# Autodesk Inventor assembly: 2021-01-001_o
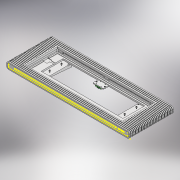
[picture p0: Inventor's stored thumbnail of the model, 180x180]
Saved by Autodesk Inventor 2020.2 (Build 242310000, 310)
## iProperties
Created: 2021-04-25
Part Number: 2021-01-001_o
Document SubType Name: Assembly
Designer: carso
Author: carso
## Documents named in this file (75)
- P:\Carson Wright Design Projects\KB__kbd-2600\KBD2600 MANUFACTURING ASSETS\CAD FILES\IPT\2021-01-001_o.iam
- P:\Carson Wright Design Projects\KB__kbd-2600\FINAL\2021-01-002.ipt
- P:\Carson Wright Design Projects\KB__kbd-2600\FINAL\2021-01-006.ipt
- P:\Carson Wright Design Projects\KB__kbd-2600\FINAL\2021-01-011.ipt
- P:\Carson Wright Design Projects\KB__kbd-2600\FINAL\2021-01-013_pp.ipt
- P:\Carson Wright Design Projects\KB__kbd-2600\FINAL\2021-01-017_pp.ipt
- P:\Carson Wright Design Projects\KB__kbd-2600\FINAL\2021-01-015_pp.ipt
- P:\Carson Wright Design Projects\KB__kbd-2600\FINAL\2021-01-003.ipt
- P:\Carson Wright Design Projects\KB__kbd-2600\FINAL\2021-01-021_pp.ipt
- P:\Carson Wright Design Projects\KB__kbd-2600\FINAL\2021-01-019_pp.ipt
- P:\Carson Wright Design Projects\KB__kbd-2600\FINAL\2021-01-018_pp.ipt
- P:\Carson Wright Design Projects\KB__kbd-2600\FINAL\2021-01-016.ipt
- P:\Carson Wright Design Projects\KB__kbd-2600\FINAL\2021-01-022.iam
- P:\Carson Wright Design Projects\KB__kbd-2600\FINAL\2021-01-020_pp.ipt
- P:\Carson Wright Design Projects\KB__kbd-2600\FINAL\2021-01-007.ipt
- P:\Carson Wright Design Projects\KB__kbd-2600\FINAL\2021-01-008.ipt
- P:\Assets\Keycaps\CherryMX-master\CherryMX-master-updated\CherryMX-master\r1 legended\STP\Esc.ipt
- P:\Assets\Keycaps\CherryMX-master\CherryMX-master-updated\CherryMX-master\r1 legended\STP\1_NEW.ipt
- P:\Assets\Keycaps\CherryMX-master\CherryMX-master-updated\CherryMX-master\r1 legended\STP\2.ipt
- P:\Assets\Keycaps\CherryMX-master\CherryMX-master-updated\CherryMX-master\r1 legended\STP\4.ipt
- P:\Assets\Keycaps\CherryMX-master\CherryMX-master-updated\CherryMX-master\r1 legended\STP\5_NEW.ipt
- P:\Assets\Keycaps\CherryMX-master\CherryMX-master-updated\CherryMX-master\r1 legended\STP\3 ansi.ipt
- P:\Assets\Keycaps\CherryMX-master\CherryMX-master-updated\CherryMX-master\r1 legended\STP\6.ipt
- P:\Assets\Keycaps\CherryMX-master\CherryMX-master-updated\CherryMX-master\r1 legended\STP\7.ipt
- P:\Assets\Keycaps\CherryMX-master\CherryMX-master-updated\CherryMX-master\r1 legended\STP\8.ipt
- P:\Assets\Keycaps\CherryMX-master\CherryMX-master-updated\CherryMX-master\r1 legended\STP\9.ipt
- P:\Assets\Keycaps\CherryMX-master\CherryMX-master-updated\CherryMX-master\r1 legended\STP\-.ipt
- P:\Assets\Keycaps\CherryMX-master\CherryMX-master-updated\CherryMX-master\r1 legended\STP\0.ipt
- P:\Assets\Keycaps\CherryMX-master\CherryMX-master-updated\CherryMX-master\r1 legended\STP\=.ipt
- P:\Assets\Keycaps\CherryMX-master\CherryMX-master-updated\CherryMX-master\r1 legended\STP\TILDE.ipt
- P:\Assets\Keycaps\CherryMX-master\CherryMX-master-updated\CherryMX-master\r1 legended\STP\pipe.ipt
- P:\Assets\Keycaps\CherryMX-master\CherryMX-master-updated\CherryMX-master\r2 legended\STP\Q.ipt
- P:\Assets\Keycaps\CherryMX-master\CherryMX-master-updated\CherryMX-master\r2 legended\STP\W.ipt
- P:\Assets\Keycaps\CherryMX-master\CherryMX-master-updated\CherryMX-master\r2 legended\STP\E.ipt
- P:\Assets\Keycaps\CherryMX-master\CherryMX-master-updated\CherryMX-master\r2 legended\STP\R.ipt
- P:\Assets\Keycaps\CherryMX-master\CherryMX-master-updated\CherryMX-master\r2 legended\STP\T.ipt
- P:\Assets\Keycaps\CherryMX-master\CherryMX-master-updated\CherryMX-master\r2 legended\STP\Y.ipt
- P:\Assets\Keycaps\CherryMX-master\CherryMX-master-updated\CherryMX-master\r2 legended\STP\U.ipt
- P:\Assets\Keycaps\CherryMX-master\CherryMX-master-updated\CherryMX-master\r2 legended\STP\I.ipt
- P:\Assets\Keycaps\CherryMX-master\CherryMX-master-updated\CherryMX-master\r2 legended\STP\O.ipt
- P:\Assets\Keycaps\CherryMX-master\CherryMX-master-updated\CherryMX-master\r2 legended\STP\P.ipt
- P:\Assets\Keycaps\CherryMX-master\CherryMX-master-updated\CherryMX-master\r2 legended\STP\OPEN BRACKETS.ipt
- P:\Assets\Keycaps\CherryMX-master\CherryMX-master-updated\CherryMX-master\r2 legended\STP\CLOSE BRACKETS.ipt
- P:\Assets\Keycaps\CherryMX-master\CherryMX-master-updated\CherryMX-master\r2 legended\STP\15\Backspace text.ipt
- P:\Assets\Keycaps\CherryMX-master\CherryMX-master-updated\CherryMX-master\r2 legended\STP\15\Tab text.ipt
- P:\Assets\Keycaps\CherryMX-master\CherryMX-master-updated\CherryMX-master\r3 legended\STP\175\Control.ipt
- P:\Assets\Keycaps\CherryMX-master\CherryMX-master-updated\CherryMX-master\r3 legended\STP\A.ipt
- P:\Assets\Keycaps\CherryMX-master\CherryMX-master-updated\CherryMX-master\r3 legended\STP\S.ipt
- P:\Assets\Keycaps\CherryMX-master\CherryMX-master-updated\CherryMX-master\r3 legended\STP\D.ipt
- P:\Assets\Keycaps\CherryMX-master\CherryMX-master-updated\CherryMX-master\r3 legended\STP\F_homing_bar.ipt
- P:\Assets\Keycaps\CherryMX-master\CherryMX-master-updated\CherryMX-master\r3 legended\STP\G.ipt
- P:\Assets\Keycaps\CherryMX-master\CherryMX-master-updated\CherryMX-master\r3 legended\STP\H.ipt
- P:\Assets\Keycaps\CherryMX-master\CherryMX-master-updated\CherryMX-master\r3 legended\STP\J_homing_bar.ipt
- P:\Assets\Keycaps\CherryMX-master\CherryMX-master-updated\CherryMX-master\r3 legended\STP\K.ipt
- P:\Assets\Keycaps\CherryMX-master\CherryMX-master-updated\CherryMX-master\r3 legended\STP\L.ipt
- P:\Assets\Keycaps\CherryMX-master\CherryMX-master-updated\CherryMX-master\r3 legended\STP\COLONS.ipt
- P:\Assets\Keycaps\CherryMX-master\CherryMX-master-updated\CherryMX-master\r3 legended\STP\quotes.ipt
- P:\Assets\Keycaps\CherryMX-master\CherryMX-master\r3 legended\STP\225\Enter Text 225 Fixed.ipt
- P:\Assets\Keycaps\CherryMX-master\CherryMX-master\r4 legended\STP\225\Shift text.ipt
- P:\Assets\Keycaps\CherryMX-master\CherryMX-master\r4 legended\STP\Z.ipt
- P:\Assets\Keycaps\CherryMX-master\CherryMX-master\r4 legended\STP\X.ipt
- P:\Assets\Keycaps\CherryMX-master\CherryMX-master\r4 legended\STP\C.ipt
- P:\Assets\Keycaps\CherryMX-master\CherryMX-master\r4 legended\STP\V.ipt
- P:\Assets\Keycaps\CherryMX-master\CherryMX-master\r4 legended\STP\B.ipt
- P:\Assets\Keycaps\CherryMX-master\CherryMX-master\r4 legended\STP\N.ipt
- P:\Assets\Keycaps\CherryMX-master\CherryMX-master\r4 legended\STP\M.ipt
- P:\Assets\Keycaps\CherryMX-master\CherryMX-master\r4 legended\STP\COMMA.ipt
- P:\Assets\Keycaps\CherryMX-master\CherryMX-master\r4 legended\STP\FULL STOP.ipt
- P:\Assets\Keycaps\CherryMX-master\CherryMX-master\r4 legended\STP\Fn.ipt
- P:\Assets\Keycaps\CherryMX-master\CherryMX-master\r4 legended\STP\FORWARD SLASH.ipt
- P:\Assets\Keycaps\CherryMX-master\CherryMX-master\r4 legended\STP\175\Shift short text.ipt
- P:\Assets\Keycaps\CherryMX-master\CherryMX-master\STEP\r4\r4_150.ipt
- P:\Assets\Keycaps\CherryMX-master\CherryMX-master-updated\CherryMX-master\r4 legended\STP\CODE.ipt
- P:\Assets\Keycaps\CherryMX-master\CherryMX-master-updated\CherryMX-master\r4 legended\STP\15\Alt.ipt
- P:\Assets\Keycaps\CherryMX-master\CherryMX-master-updated\CherryMX-master\STEP\r4\r4_700.ipt
## Components (102 placed, 74 different names)
1. 2021-01-002:1 — Mate:34, Mate:35, Mate:36, Mate:37, Mate:38, Mate:39, Mate:40, Mate:41, Mate:42, Mate:43, Mate:44, Mate:45, Mate:53, Mate:54, Mate:55, Mate:57, Mate:59, Mate:61, Mate:63, Mate:65, Mate:67, Mate:68, Mate:69, Mate:70, Mate:71, Mate:73, Mate:75, Mate:77, Mate:79, Mate:80, Mate:81, Mate:82, Mate:83, Mate:84, Mate:85, Mate:86, Mate:87, Mate:88, Mate:89, Mate:90
2. 2021-01-006:1 — Mate:46, Mate:47, Mate:48, Mate:49, Mate:51, Mate:68, Mate:69, Mate:70, Mate:116, Mate:117, Mate:118, Mate:119
3. 2021-01-011:1 — Mate:4, Mate:5, Mate:6, Mate:46, Mate:47, Mate:48, Mate:50, Mate:52
4. 2021-01-013_pp:1 — Mate:4, Mate:5, Mate:6, Mate:7, Mate:8, Mate:9, Mate:10, Mate:11, Mate:12, Mate:13, Mate:14
5. 2021-01-017_pp:1 — Mate:7, Mate:8
6. 2021-01-017_pp:2 — Mate:9, Mate:10
7. 2021-01-017_pp:3 — Mate:13, Mate:14
8. 2021-01-017_pp:4 — Mate:11, Mate:12
9. 2021-01-015_pp:1 — Mate:34, Mate:35, Mate:36
10. 2021-01-015_pp:2 — Mate:37, Mate:38, Mate:39
11. 2021-01-015_pp:3 — Mate:43, Mate:44, Mate:45
12. 2021-01-015_pp:4 — Mate:40, Mate:41, Mate:42
13. 2021-01-003:1 — Mate:53, Mate:54, Mate:55, Mate:56, Mate:58, Mate:60, Mate:62, Mate:64, Mate:66, Mate:92, Mate:93, Mate:94, Mate:95, Mate:96, Mate:97, Mate:98, Mate:99, Mate:100, Mate:101, Mate:110, Mate:111, Mate:112, Mate:113, Mate:114, Mate:115
14. 2021-01-021_pp:1 — Mate:51, Mate:52
15. 2021-01-021_pp:2 — Mate:49, Mate:50
16. 2021-01-019_pp:1 — Mate:58, Mate:59
17. 2021-01-019_pp:2 — Mate:56, Mate:57
18. 2021-01-019_pp:3 — Mate:66, Mate:67
19. 2021-01-019_pp:4 — Mate:64, Mate:65
20. 2021-01-019_pp:5 — Mate:60, Mate:61
21. 2021-01-019_pp:6 — Mate:62, Mate:63
22. 2021-01-018_pp:1 — Mate:71, Mate:116
23. 2021-01-018_pp:2 — Mate:73, Mate:117
24. 2021-01-018_pp:3 — Mate:75, Mate:118
25. 2021-01-018_pp:4 — Mate:77, Mate:119
26. 2021-01-016:1 — Mate:88, Mate:89, Mate:90
27. 2021-01-016:2 — Mate:82, Mate:83, Mate:84
28. 2021-01-016:3 — Mate:79, Mate:80, Mate:81
29. 2021-01-016:4 — Mate:85, Mate:86, Mate:87, Mate:91
30. 2021-01-022:1 [sub-assembly] — Mate:91, Mate:92, Mate:93, Mate:120, Mate:121, Mate:122, Mate:123, Mate:124, Mate:125, Mate:128, Mate:129, Mate:130, Mate:131, Mate:132, Mate:133, Mate:134, Mate:135, Mate:136, Mate:137, Mate:138, Mate:139, Mate:140, Mate:141, Mate:142, Mate:143, Mate:144, Mate:145, Mate:146, Mate:147, Mate:148, Mate:149, Mate:150, Mate:151, Mate:154, Mate:155, Mate:156, Mate:157, Mate:158, Mate:159, Mate:160, Mate:161, Mate:162, Mate:163, Mate:164, Mate:165, Mate:166, Mate:167, Mate:168, Mate:169, Mate:170, Mate:171, Mate:172, Mate:173, Mate:174, Mate:175, Mate:176, Mate:177, Mate:178, Mate:179, Mate:180, Mate:181, Mate:182, Mate:183, Mate:184, Mate:185, Mate:186, Mate:187, Mate:188, Mate:189, Mate:190, Mate:191, Mate:192, Mate:193, Mate:194, Mate:195, Mate:196, Mate:197, Mate:198, Mate:199, Mate:200, Mate:201, Mate:202, Mate:203, Mate:204, Mate:205, Mate:206, Mate:207, Mate:208, Mate:209, Mate:210, Mate:211, Mate:212, Mate:213, Mate:214, Mate:215, Mate:216, Mate:217, Mate:218, Mate:219, Mate:220, Mate:221, Mate:222, Mate:223, Mate:224, Mate:225, Mate:226, Mate:227, Mate:228, Mate:229, Mate:230, Mate:231, Mate:232, Mate:233, Mate:234, Mate:235, Mate:236, Mate:237, Mate:238, Mate:239, Mate:240, Mate:241, Mate:242, Mate:243, Mate:244, Mate:245, Mate:246, Mate:247
31. 2021-01-020_pp:1 — Mate:94, Mate:95
32. 2021-01-020_pp:2 — Mate:96, Mate:97
33. 2021-01-020_pp:3 — Mate:100, Mate:101
34. 2021-01-020_pp:4 — Mate:98, Mate:99
35. 2021-01-007:1 — Mate:106, Mate:107, Mate:108, Mate:109, Mate:113, Mate:114, Mate:115
36. 2021-01-008:1 — Mate:102, Mate:103, Mate:104, Mate:105, Mate:110, Mate:111, Mate:112
37. 2021-01-020_pp:5 — Mate:102, Mate:103
38. 2021-01-020_pp:6 — Mate:108, Mate:109
39. 2021-01-020_pp:7 — Mate:106, Mate:107
40. 2021-01-020_pp:8 — Mate:104, Mate:105
41. Esc:1 — Mate:120, Mate:121
42. 1_NEW:1 — Mate:122, Mate:123
43. 2:1 — Mate:124, Mate:125
44. 4:1 — Mate:128, Mate:129
45. 5_NEW:1 — Mate:132, Mate:133
46. 3 ansi:1 — Mate:130, Mate:131
47. 6:1 — Mate:134, Mate:135
48. 7:1 — Mate:136, Mate:137
49. 8:1 — Mate:138, Mate:139
50. 9:1 — Mate:140, Mate:141
51. -:1 — Mate:144, Mate:145
52. 0:1 — Mate:142, Mate:143
53. =:1 — Mate:146, Mate:147
54. TILDE:1 — Mate:150, Mate:151
55. pipe:1 — Mate:148, Mate:149
56. Q:1 — Mate:154, Mate:155
57. W:1 — Mate:156, Mate:157
58. E:1 — Mate:158, Mate:159
59. R:1 — Mate:160, Mate:161
60. T:1 — Mate:162, Mate:163
61. Y:1 — Mate:164, Mate:165
62. U:1 — Mate:166, Mate:167
63. I:1 — Mate:168, Mate:169
64. O:1 — Mate:170, Mate:171
65. P:1 — Mate:172, Mate:173
66. OPEN BRACKETS:1 — Mate:174, Mate:175
67. CLOSE BRACKETS:1 — Mate:176, Mate:177
68. Backspace text:1 — Mate:178, Mate:179
69. Tab text:1 — Mate:180, Mate:181
70. Control:1 — Mate:182, Mate:183
71. A:1 — Mate:184, Mate:185
72. S:1 — Mate:186, Mate:187
73. D:1 — Mate:188, Mate:189
74. F_homing_bar:1 — Mate:190, Mate:191
75. G:1 — Mate:192, Mate:193
76. H:1 — Mate:194, Mate:195
77. J_homing_bar:1 — Mate:196, Mate:197
78. K:1 — Mate:198, Mate:199
79. L:1 — Mate:200, Mate:201
80. COLONS:1 — Mate:202, Mate:203
81. quotes:1 — Mate:204, Mate:205
82. Enter Text 225 Fixed:1 — Mate:206, Mate:207
83. Shift text:1 — Mate:208, Mate:209
84. Z:1 — Mate:210, Mate:211
85. X:1 — Mate:212, Mate:213
86. C:1 — Mate:214, Mate:215
87. V:1 — Mate:216, Mate:217
88. B:1 — Mate:218, Mate:219
89. N:1 — Mate:222, Mate:223
90. M:1 — Mate:220, Mate:221
91. COMMA:1 — Mate:224, Mate:225
92. FULL STOP:1 — Mate:226, Mate:227
93. Fn:1 — Mate:230, Mate:231
94. FORWARD SLASH:1 — Mate:228, Mate:229
95. Shift short text:1 — Mate:232, Mate:233
96. r4_150:1 — Mate:234, Mate:235
97. r4_150:2 — Mate:236, Mate:237
98. CODE:1 — Mate:238, Mate:239
99. CODE:2 — Mate:240, Mate:241
100. Alt:1 — Mate:242, Mate:243
101. Alt:2 — Mate:244, Mate:245
102. r4_700:1 — Mate:246, Mate:247
## Relationships (217: Mate 217)
- Mate:4: 2021-01-011:1 ↔ 2021-01-013_pp:1
- Mate:5: 2021-01-011:1 ↔ 2021-01-013_pp:1
- Mate:6: 2021-01-011:1 ↔ 2021-01-013_pp:1
- Mate:7: 2021-01-013_pp:1 ↔ 2021-01-017_pp:1
- Mate:8: 2021-01-013_pp:1 ↔ 2021-01-017_pp:1
- Mate:9: 2021-01-013_pp:1 ↔ 2021-01-017_pp:2
- Mate:10: 2021-01-013_pp:1 ↔ 2021-01-017_pp:2
- Mate:11: 2021-01-013_pp:1 ↔ 2021-01-017_pp:4
- Mate:12: 2021-01-013_pp:1 ↔ 2021-01-017_pp:4
- Mate:13: 2021-01-013_pp:1 ↔ 2021-01-017_pp:3
- Mate:14: 2021-01-013_pp:1 ↔ 2021-01-017_pp:3
- Mate:34 (0.1 mm): 2021-01-002:1 ↔ 2021-01-015_pp:1
- Mate:35: 2021-01-002:1 ↔ 2021-01-015_pp:1
- Mate:36: 2021-01-002:1 ↔ 2021-01-015_pp:1
- Mate:37 (0.1 mm): 2021-01-002:1 ↔ 2021-01-015_pp:2
- Mate:38: 2021-01-002:1 ↔ 2021-01-015_pp:2
- Mate:39: 2021-01-002:1 ↔ 2021-01-015_pp:2
- Mate:40 (0.1 mm): 2021-01-002:1 ↔ 2021-01-015_pp:4
- Mate:41: 2021-01-002:1 ↔ 2021-01-015_pp:4
- Mate:42: 2021-01-002:1 ↔ 2021-01-015_pp:4
- Mate:43 (0.1 mm): 2021-01-002:1 ↔ 2021-01-015_pp:3
- Mate:44: 2021-01-002:1 ↔ 2021-01-015_pp:3
- Mate:45: 2021-01-002:1 ↔ 2021-01-015_pp:3
- Mate:46: 2021-01-006:1 ↔ 2021-01-011:1
- Mate:47: 2021-01-006:1 ↔ 2021-01-011:1
- Mate:48: 2021-01-006:1 ↔ 2021-01-011:1
- Mate:49: 2021-01-006:1 ↔ 2021-01-021_pp:2
- Mate:50: 2021-01-011:1 ↔ 2021-01-021_pp:2
- Mate:51: 2021-01-006:1 ↔ 2021-01-021_pp:1
- Mate:52: 2021-01-011:1 ↔ 2021-01-021_pp:1
- Mate:53: 2021-01-002:1 ↔ 2021-01-003:1
- Mate:54: 2021-01-002:1 ↔ 2021-01-003:1
- Mate:55: 2021-01-002:1 ↔ 2021-01-003:1
- Mate:56: 2021-01-003:1 ↔ 2021-01-019_pp:2
- Mate:57: 2021-01-002:1 ↔ 2021-01-019_pp:2
- Mate:58: 2021-01-003:1 ↔ 2021-01-019_pp:1
- Mate:59: 2021-01-002:1 ↔ 2021-01-019_pp:1
- Mate:60: 2021-01-003:1 ↔ 2021-01-019_pp:5
- Mate:61: 2021-01-002:1 ↔ 2021-01-019_pp:5
- Mate:62: 2021-01-003:1 ↔ 2021-01-019_pp:6
- Mate:63: 2021-01-002:1 ↔ 2021-01-019_pp:6
- Mate:64: 2021-01-003:1 ↔ 2021-01-019_pp:4
- Mate:65: 2021-01-002:1 ↔ 2021-01-019_pp:4
- Mate:66: 2021-01-003:1 ↔ 2021-01-019_pp:3
- Mate:67: 2021-01-002:1 ↔ 2021-01-019_pp:3
- Mate:68: 2021-01-002:1 ↔ 2021-01-006:1
- Mate:69: 2021-01-002:1 ↔ 2021-01-006:1
- Mate:70: 2021-01-002:1 ↔ 2021-01-006:1
- Mate:71: 2021-01-002:1 ↔ 2021-01-018_pp:1
- Mate:73: 2021-01-002:1 ↔ 2021-01-018_pp:2
- Mate:75: 2021-01-002:1 ↔ 2021-01-018_pp:3
- Mate:77: 2021-01-002:1 ↔ 2021-01-018_pp:4
- Mate:79: 2021-01-002:1 ↔ 2021-01-016:3
- Mate:80: 2021-01-002:1 ↔ 2021-01-016:3
- Mate:81: 2021-01-002:1 ↔ 2021-01-016:3
- Mate:82: 2021-01-002:1 ↔ 2021-01-016:2
- Mate:83: 2021-01-002:1 ↔ 2021-01-016:2
- Mate:84: 2021-01-002:1 ↔ 2021-01-016:2
- Mate:85: 2021-01-002:1 ↔ 2021-01-016:4
- Mate:86: 2021-01-002:1 ↔ 2021-01-016:4
- Mate:87: 2021-01-002:1 ↔ 2021-01-016:4
- Mate:88: 2021-01-002:1 ↔ 2021-01-016:1
- Mate:89: 2021-01-002:1 ↔ 2021-01-016:1
- Mate:90: 2021-01-002:1 ↔ 2021-01-016:1
- Mate:91: 2021-01-016:4 ↔ 2021-01-022:1
- Mate:92 (0.2 mm): 2021-01-003:1 ↔ 2021-01-022:1
- Mate:93 (0.2 mm): 2021-01-003:1 ↔ 2021-01-022:1
- Mate:94: 2021-01-003:1 ↔ 2021-01-020_pp:1
- Mate:95: 2021-01-003:1 ↔ 2021-01-020_pp:1
- Mate:96: 2021-01-003:1 ↔ 2021-01-020_pp:2
- Mate:97: 2021-01-003:1 ↔ 2021-01-020_pp:2
- Mate:98: 2021-01-003:1 ↔ 2021-01-020_pp:4
- Mate:99: 2021-01-003:1 ↔ 2021-01-020_pp:4
- Mate:100: 2021-01-003:1 ↔ 2021-01-020_pp:3
- Mate:101: 2021-01-003:1 ↔ 2021-01-020_pp:3
- Mate:102: 2021-01-008:1 ↔ 2021-01-020_pp:5
- Mate:103: 2021-01-008:1 ↔ 2021-01-020_pp:5
- Mate:104: 2021-01-008:1 ↔ 2021-01-020_pp:8
- Mate:105: 2021-01-008:1 ↔ 2021-01-020_pp:8
- Mate:106: 2021-01-007:1 ↔ 2021-01-020_pp:7
- Mate:107: 2021-01-007:1 ↔ 2021-01-020_pp:7
- Mate:108: 2021-01-007:1 ↔ 2021-01-020_pp:6
- Mate:109: 2021-01-007:1 ↔ 2021-01-020_pp:6
- Mate:110 (0.2 mm): 2021-01-003:1 ↔ 2021-01-008:1
- Mate:111 (0.2 mm): 2021-01-003:1 ↔ 2021-01-008:1
- Mate:112: 2021-01-003:1 ↔ 2021-01-008:1
- Mate:113 (0.2 mm): 2021-01-003:1 ↔ 2021-01-007:1
- Mate:114 (0.2 mm): 2021-01-003:1 ↔ 2021-01-007:1
- Mate:115: 2021-01-003:1 ↔ 2021-01-007:1
- Mate:116: 2021-01-006:1 ↔ 2021-01-018_pp:1
- Mate:117: 2021-01-006:1 ↔ 2021-01-018_pp:2
- Mate:118: 2021-01-006:1 ↔ 2021-01-018_pp:3
- Mate:119: 2021-01-006:1 ↔ 2021-01-018_pp:4
- Mate:120: 2021-01-022:1 ↔ Esc:1
- Mate:121: 2021-01-022:1 ↔ Esc:1
- Mate:122: 2021-01-022:1 ↔ 1_NEW:1
- Mate:123: 2021-01-022:1 ↔ 1_NEW:1
- Mate:124: 2021-01-022:1 ↔ 2:1
- Mate:125: 2021-01-022:1 ↔ 2:1
- Mate:128: 2021-01-022:1 ↔ 4:1
- Mate:129: 2021-01-022:1 ↔ 4:1
- Mate:130: 2021-01-022:1 ↔ 3 ansi:1
- Mate:131: 2021-01-022:1 ↔ 3 ansi:1
- Mate:132: 2021-01-022:1 ↔ 5_NEW:1
- Mate:133: 2021-01-022:1 ↔ 5_NEW:1
- Mate:134: 2021-01-022:1 ↔ 6:1
- Mate:135: 2021-01-022:1 ↔ 6:1
- Mate:136: 2021-01-022:1 ↔ 7:1
- Mate:137: 2021-01-022:1 ↔ 7:1
- Mate:138: 2021-01-022:1 ↔ 8:1
- Mate:139: 2021-01-022:1 ↔ 8:1
- Mate:140: 2021-01-022:1 ↔ 9:1
- Mate:141: 2021-01-022:1 ↔ 9:1
- Mate:142: 2021-01-022:1 ↔ 0:1
- Mate:143: 2021-01-022:1 ↔ 0:1
- Mate:144: 2021-01-022:1 ↔ -:1
- Mate:145: 2021-01-022:1 ↔ -:1
- Mate:146: 2021-01-022:1 ↔ =:1
- Mate:147: 2021-01-022:1 ↔ =:1
- Mate:148: 2021-01-022:1 ↔ pipe:1
- Mate:149: 2021-01-022:1 ↔ pipe:1
- Mate:150: 2021-01-022:1 ↔ TILDE:1
- Mate:151: 2021-01-022:1 ↔ TILDE:1
- Mate:154: 2021-01-022:1 ↔ Q:1
- Mate:155: 2021-01-022:1 ↔ Q:1
- Mate:156: 2021-01-022:1 ↔ W:1
- Mate:157: 2021-01-022:1 ↔ W:1
- Mate:158: 2021-01-022:1 ↔ E:1
- Mate:159: 2021-01-022:1 ↔ E:1
- Mate:160: 2021-01-022:1 ↔ R:1
- Mate:161: 2021-01-022:1 ↔ R:1
- Mate:162: 2021-01-022:1 ↔ T:1
- Mate:163: 2021-01-022:1 ↔ T:1
- Mate:164: 2021-01-022:1 ↔ Y:1
- Mate:165: 2021-01-022:1 ↔ Y:1
- Mate:166: 2021-01-022:1 ↔ U:1
- Mate:167: 2021-01-022:1 ↔ U:1
- Mate:168: 2021-01-022:1 ↔ I:1
- Mate:169: 2021-01-022:1 ↔ I:1
- Mate:170: 2021-01-022:1 ↔ O:1
- Mate:171: 2021-01-022:1 ↔ O:1
- Mate:172: 2021-01-022:1 ↔ P:1
- Mate:173: 2021-01-022:1 ↔ P:1
- Mate:174: 2021-01-022:1 ↔ OPEN BRACKETS:1
- Mate:175: 2021-01-022:1 ↔ OPEN BRACKETS:1
- Mate:176: 2021-01-022:1 ↔ CLOSE BRACKETS:1
- Mate:177: 2021-01-022:1 ↔ CLOSE BRACKETS:1
- Mate:178: 2021-01-022:1 ↔ Backspace text:1
- Mate:179: 2021-01-022:1 ↔ Backspace text:1
- Mate:180: 2021-01-022:1 ↔ Tab text:1
- Mate:181: 2021-01-022:1 ↔ Tab text:1
- Mate:182: 2021-01-022:1 ↔ Control:1
- Mate:183: 2021-01-022:1 ↔ Control:1
- Mate:184: 2021-01-022:1 ↔ A:1
- Mate:185: 2021-01-022:1 ↔ A:1
- Mate:186: 2021-01-022:1 ↔ S:1
- Mate:187: 2021-01-022:1 ↔ S:1
- Mate:188: 2021-01-022:1 ↔ D:1
- Mate:189: 2021-01-022:1 ↔ D:1
- Mate:190: 2021-01-022:1 ↔ F_homing_bar:1
- Mate:191: 2021-01-022:1 ↔ F_homing_bar:1
- Mate:192: 2021-01-022:1 ↔ G:1
- Mate:193: 2021-01-022:1 ↔ G:1
- Mate:194: 2021-01-022:1 ↔ H:1
- Mate:195: 2021-01-022:1 ↔ H:1
- Mate:196: 2021-01-022:1 ↔ J_homing_bar:1
- Mate:197: 2021-01-022:1 ↔ J_homing_bar:1
- Mate:198: 2021-01-022:1 ↔ K:1
- Mate:199: 2021-01-022:1 ↔ K:1
- Mate:200: 2021-01-022:1 ↔ L:1
- Mate:201: 2021-01-022:1 ↔ L:1
- Mate:202: 2021-01-022:1 ↔ COLONS:1
- Mate:203: 2021-01-022:1 ↔ COLONS:1
- Mate:204: 2021-01-022:1 ↔ quotes:1
- Mate:205: 2021-01-022:1 ↔ quotes:1
- Mate:206: 2021-01-022:1 ↔ Enter Text 225 Fixed:1
- Mate:207: 2021-01-022:1 ↔ Enter Text 225 Fixed:1
- Mate:208: 2021-01-022:1 ↔ Shift text:1
- Mate:209: 2021-01-022:1 ↔ Shift text:1
- Mate:210: 2021-01-022:1 ↔ Z:1
- Mate:211: 2021-01-022:1 ↔ Z:1
- Mate:212: 2021-01-022:1 ↔ X:1
- Mate:213: 2021-01-022:1 ↔ X:1
- Mate:214: 2021-01-022:1 ↔ C:1
- Mate:215: 2021-01-022:1 ↔ C:1
- Mate:216: 2021-01-022:1 ↔ V:1
- Mate:217: 2021-01-022:1 ↔ V:1
- Mate:218: 2021-01-022:1 ↔ B:1
- Mate:219: 2021-01-022:1 ↔ B:1
- Mate:220: 2021-01-022:1 ↔ M:1
- Mate:221: 2021-01-022:1 ↔ M:1
- Mate:222: 2021-01-022:1 ↔ N:1
- Mate:223: 2021-01-022:1 ↔ N:1
- Mate:224: 2021-01-022:1 ↔ COMMA:1
- Mate:225: 2021-01-022:1 ↔ COMMA:1
- Mate:226: 2021-01-022:1 ↔ FULL STOP:1
- Mate:227: 2021-01-022:1 ↔ FULL STOP:1
- Mate:228: 2021-01-022:1 ↔ FORWARD SLASH:1
- Mate:229: 2021-01-022:1 ↔ FORWARD SLASH:1
- Mate:230: 2021-01-022:1 ↔ Fn:1
- Mate:231: 2021-01-022:1 ↔ Fn:1
- Mate:232: 2021-01-022:1 ↔ Shift short text:1
- Mate:233: 2021-01-022:1 ↔ Shift short text:1
- Mate:234: 2021-01-022:1 ↔ r4_150:1
- Mate:235: 2021-01-022:1 ↔ r4_150:1
- Mate:236: 2021-01-022:1 ↔ r4_150:2
- Mate:237: 2021-01-022:1 ↔ r4_150:2
- Mate:238: 2021-01-022:1 ↔ CODE:1
- Mate:239: 2021-01-022:1 ↔ CODE:1
- Mate:240: 2021-01-022:1 ↔ CODE:2
- Mate:241: 2021-01-022:1 ↔ CODE:2
- Mate:242: 2021-01-022:1 ↔ Alt:1
- Mate:243: 2021-01-022:1 ↔ Alt:1
- Mate:244: 2021-01-022:1 ↔ Alt:2
- Mate:245: 2021-01-022:1 ↔ Alt:2
- Mate:246: 2021-01-022:1 ↔ r4_700:1
- Mate:247: 2021-01-022:1 ↔ r4_700:1
